# Autodesk Inventor assembly: brace
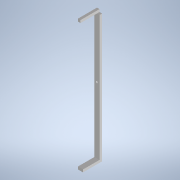
[picture p0: Inventor's stored thumbnail of the model, 180x180]
Saved by Autodesk Inventor 2020.2 (Build 242310000, 310)
## iProperties
Created: 2020-02-12
Part Number: brace
Document SubType Name: Assembly
Designer: ColinP
Author: ColinP
## Documents named in this file (3)
- C:\Users\ColinP\Documents\Inventor\steppermotoriqc\brace.iam
- C:\Users\ColinP\Documents\Inventor\steppermotoriqc\brace1.ipt
- C:\Users\ColinP\Documents\Inventor\steppermotoriqc\brace2.ipt
## Components (2 placed, 2 different names)
1. brace1:1 — Mate:2, Flush:1, Mate:3, Flush:2
2. brace2:1 — Mate:2, Flush:1, Mate:3, Flush:2
## Relationships (4: Mate 2, Flush 2)
- Mate:2: brace1:1 ↔ brace2:1
- Flush:1: brace1:1 ↔ brace2:1
- Mate:3: brace1:1 ↔ brace2:1
- Flush:2: brace1:1 ↔ brace2:1
